# Autodesk Inventor assembly: OBG-Antrieb
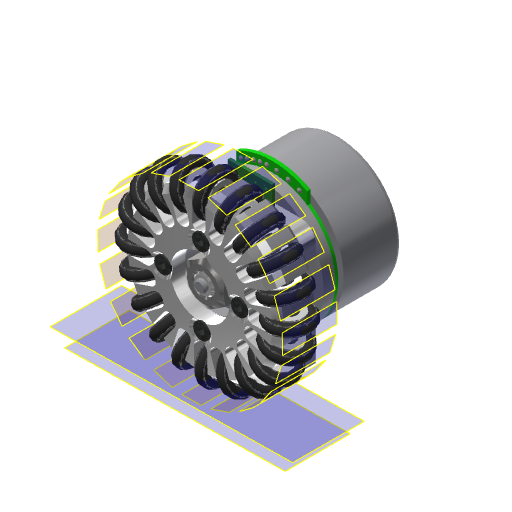
[picture p0: Inventor's stored thumbnail of the model, 512x512]
Saved by Autodesk Inventor 2022.1 (Build 261234020, 234B)
## iProperties
Part Number: OBG-Antrieb
Material: Generisch
Document SubType Name: Assembly
Designer: rYan
Mass: 234.467 g
Surface Area: 734.726 cm^2
Volume: 67.3795 cm^3
Density: 3.4798 g/cm^3
Author: rYan
## Documents named in this file (10)
- D:\TIGERsGIT\Hardware\mechanik\2020\Inventor\Robot\Drive Train\OBG-Antrieb.iam
- D:\TIGERsGIT\Hardware\mechanik\2020\Inventor\Robot\Drive Train\Lagerbock.ipt
- D:\TIGERsGIT\Hardware\mechanik\2020\Inventor\Purchased Parts\DF45L024048\DF45L024048-A2.iam
- D:\TIGERsGIT\Hardware\mechanik\2020\Inventor\Inhaltscenter\de-DE\ISO 10642(1)\ISO 10642 - M3 x  8.ipt
- D:\TIGERsGIT\Hardware\mechanik\2020\Inventor\Robot\Drive Train\UBG-Rad.iam
- D:\TIGERsGIT\Hardware\mechanik\2020\Inventor\Robot\Drive Train\MG-Encoderplatine.iam
- D:\TIGERsGIT\Hardware\mechanik\2020\Inventor\Inhaltscenter\de-DE\ISO 1580\ISO 1580 - M2 x 3.ipt
- D:\TIGERsGIT\Hardware\mechanik\2020\Inventor\Robot\Drive Train\Radadapter.ipt
- D:\TIGERsGIT\Hardware\mechanik\2020\Inventor\Inhaltscenter\de-DE\DIN 934\DIN 934 - M8 x 1,25.ipt
- D:\TIGERsGIT\Hardware\mechanik\2020\Inventor\Inhaltscenter\de-DE\DIN 137\DIN 137 - B8.ipt
## Components (12 placed, 9 different names)
1. Lagerbock:1 — Passend:24, Passend:25, Passend:26, Einfügen:1, Einfügen:2, Einfügen:3, Passend:49, Einfügen:4, Passend:56
2. DF45L024048-A2:1 [sub-assembly] — Passend:24, Passend:25, Passend:26, Passend:47, Passend:51
3. ISO 10642 M3 x  8:1 — Einfügen:1
4. ISO 10642 M3 x  8:2 — Einfügen:2
5. ISO 10642 M3 x  8:3 — Einfügen:3
6. UBG-Rad:1 [sub-assembly] — Passend:47, Passend:52, Winkel:1, Passend:54, Passend:56, Passend:58
7. MG-Encoderplatine:1 [sub-assembly] — Passend:49, Einfügen:4, Einfügen:5, Einfügen:6
8. ISO 1580 M2 x 3:1 — Einfügen:5
9. ISO 1580 M2 x 3:2 — Einfügen:6
10. Radadapter:1 — Passend:51, Passend:52, Winkel:1, Passend:54, Passend:57, Passend:59
11. DIN 934 - ersetzt durch DIN EN 24032/28673/28674 M8:1 — Passend:59, Passend:60
12. DIN 137 B8:1 — Passend:57, Passend:58, Passend:60
## Relationships (20: Mate 13, Insert 6, Angle 1)
- Passend:24 [Mate]: Lagerbock:1 ↔ DF45L024048-A2:1
- Passend:25 [Mate]: Lagerbock:1 ↔ DF45L024048-A2:1
- Passend:26 [Mate]: Lagerbock:1 ↔ DF45L024048-A2:1
- Einfügen:1 [Insert]: Lagerbock:1 ↔ ISO 10642 M3 x  8:1
- Einfügen:2 [Insert]: Lagerbock:1 ↔ ISO 10642 M3 x  8:2
- Einfügen:3 [Insert]: Lagerbock:1 ↔ ISO 10642 M3 x  8:3
- Passend:47 [Mate]: DF45L024048-A2:1 ↔ UBG-Rad:1
- Passend:49 [Mate]: Lagerbock:1 ↔ MG-Encoderplatine:1
- Einfügen:4 [Insert]: Lagerbock:1 ↔ MG-Encoderplatine:1
- Einfügen:5 [Insert]: MG-Encoderplatine:1 ↔ ISO 1580 M2 x 3:1
- Einfügen:6 [Insert]: MG-Encoderplatine:1 ↔ ISO 1580 M2 x 3:2
- Passend:51 [Mate]: DF45L024048-A2:1 ↔ Radadapter:1
- Passend:52 [Mate]: UBG-Rad:1 ↔ Radadapter:1
- Winkel:1 [Angle] (0 deg): UBG-Rad:1 ↔ Radadapter:1
- Passend:54 [Mate]: UBG-Rad:1 ↔ Radadapter:1
- Passend:56 [Mate] (0.9 mm): Lagerbock:1 ↔ UBG-Rad:1
- Passend:57 [Mate]: Radadapter:1 ↔ DIN 137 B8:1
- Passend:58 [Mate]: UBG-Rad:1 ↔ DIN 137 B8:1
- Passend:59 [Mate]: Radadapter:1 ↔ DIN 934 - ersetzt durch DIN EN 24032/28673/28674 M8:1
- Passend:60 [Mate]: DIN 934 - ersetzt durch DIN EN 24032/28673/28674 M8:1 ↔ DIN 137 B8:1
